# Autodesk Inventor assembly: foot
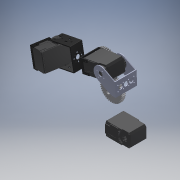
[picture p0: Inventor's stored thumbnail of the model, 180x180]
Saved by Autodesk Inventor 2019 (Build 230136000, 136)
## iProperties
Created: 2019-02-08
Part Number: foot
Document SubType Name: Assembly
Designer: mashi
Author: mashi
## iProperties of the stored document 2662N420_PLASTIC GEAR - 20 DEGREE PRESSURE ANGLE.ipt
Created: 2018-08-15
Part Number: 2662N420_PLASTIC GEAR - 20 DEGREE PRESSURE ANGLE
Material: Generic
Document SubType Name: Modeling
Designer: mashi
Density: 1 g/cm^3
Appearance: Default
Sending System: SolidWorks 2014
Last Author: T7SXC
Last Saved: 2018-08-20
Desc1: Plastic Gear—20°
Desc2: Pressure Angle
Desc3: © 2018 McMaster-Carr Supply Company
CAD Model Disclaimer and Use Terms: CAD Model Disclaimer and Use Terms.  The 3-D CAD models and related information are provided for reference only.  Your use of the CAD models is at your own risk and McMaster-Carr shall have no liability for such use.  McMaster-Carr makes no representation or warranty (express or implied) with respect to the CAD Models.  In addition, by downloading and/or using the CAD models, you agree to McMaster-Carr’s Terms and Conditions of Use and Sale, available at our website as follows: https://www.mcmaster.com/#termsandconditions
Author: mashi
## iProperties of the stored document bracketadapter2.ipt
Created: 2018-10-09
Part Number: bracketadapter2
Material: Generic
Document SubType Name: Modeling
Designer: mashi
Density: 1 g/cm^3
Appearance: Default
Sending System: SolidWorks 2018
Last Author: chang
Last Saved: 2018-10-09
Author: mashi
## iProperties of the stored document 90 Degree Servo Bracket.ipt
Created: 2018-10-07
Part Number: 90 Degree Servo Bracket
Material: Generic
Document SubType Name: Modeling
Designer: mashi
Density: 1 g/cm^3
Appearance: Default
Sending System: SolidWorks 2016
Last Author: henri
Last Saved: 2018-10-07
Author: mashi
## iProperties of the stored document Servo Motor Front Bracket.ipt
Created: 2018-10-07
Part Number: Servo Motor Front Bracket
Material: Generic
Document SubType Name: Modeling
Designer: mashi
Density: 1 g/cm^3
Appearance: Default
Sending System: SolidWorks 2018
Last Author: HP
Last Saved: 2018-10-09
Author: mashi
## iProperties of the stored document 45 Degree Servo Bracket.ipt
Created: 2018-09-28
Part Number: 45 Degree Servo Bracket
Material: Generic
Document SubType Name: Modeling
Designer: mashi
Density: 1 g/cm^3
Appearance: Default
Sending System: SolidWorks 2018
Last Author: yz3400
Last Saved: 2018-10-12
Author: mashi
## iProperties of the stored document Lewansoul LX-16A Servo.ipt
Created: 2018-10-09
Part Number: Lewansoul LX-16A Servo
Material: Generic
Description: Rhino converted to STEP
Document SubType Name: Modeling
Designer: mashi
Density: 1 g/cm^3
Appearance: Default
Sending System: SolidWorks 2018
Last Author: chang
Last Saved: 2018-10-09
Nomenclature: Document
Part Number: Document
Source: MADE
Definition: A
Author: mashi
Revision Number: A
## iProperties of the stored document Servo Motor Side Bracket.ipt
Created: 2018-10-08
Part Number: Servo Motor Side Bracket
Material: Generic
Document SubType Name: Modeling
Designer: mashi
Density: 1 g/cm^3
Appearance: Default
Sending System: SolidWorks 2018
Last Author: admin
Last Saved: 2018-10-08
Author: mashi
## iProperties of the stored document bracketadapter1.ipt
Created: 2018-10-09
Part Number: bracketadapter1
Material: Generic
Document SubType Name: Modeling
Designer: mashi
Density: 1 g/cm^3
Appearance: Default
Sending System: SolidWorks 2018
Last Author: chang
Last Saved: 2018-10-26
Author: mashi
## Documents named in this file (17)
- **C:\Users\mashi\Desktop\Robotics Studio\Rollbot\foot.iam*LocalDocs*xMgcmj2lsNkefe0wdXyyahf42Mc*2662N420_PLASTIC GEAR - 20 DEGREE PRESSURE ANGLE.ipt
- **C:\Users\mashi\Desktop\Robotics Studio\Rollbot\foot.iam*LocalDocs*x5lasmzqhNc3iev4mMcwajm4oAd*bracketadapter2.ipt
- **C:\Users\mashi\Desktop\Robotics Studio\Rollbot\foot.iam*LocalDocs*x1hcrqoyvZnlvu3kpF2lxyrgt4f*90 Degree Servo Bracket.ipt
- **C:\Users\mashi\Desktop\Robotics Studio\Rollbot\foot.iam*LocalDocs*xLrj4xvnuB5roujkdXhhuxaueNh*Servo Motor Front Bracket.ipt
- **C:\Users\mashi\Desktop\Robotics Studio\Rollbot\foot.iam*LocalDocs*xTrqjmq2aYiq3umchNmrlfejoAg*45 Degree Servo Bracket.ipt
- **C:\Users\mashi\Desktop\Robotics Studio\Rollbot\foot.iam*LocalDocs*xRjd4zsbt1wuze3ohJqu54l3rWh*Lewansoul LX-16A Servo.ipt
- **C:\Users\mashi\Desktop\Robotics Studio\Rollbot\foot.iam*LocalDocs*xVpqaq2tw5ebsussnJvcm3i000d*Servo Motor Side Bracket.ipt
- **C:\Users\mashi\Desktop\Robotics Studio\Rollbot\foot.iam*LocalDocs*xWucropqwTi4ve1g5An43dijzIb*bracketadapter1.ipt
- C:\Users\mashi\Desktop\Robotics Studio\Rollbot\foot.iam
- C:\Users\mashi\Desktop\Robotics Studio\Robotics Studio___CAD Models of Electronic Components\Lewansoul LX-16A Servo.SLDPRT
- C:\Users\mashi\Desktop\Robotics Studio\Robotics Studio___CAD Models of Electronic Components\bracketadapter1.SLDPRT
- C:\Users\mashi\Desktop\Robotics Studio\Robotics Studio___CAD Models of Electronic Components\bracketadapter2.SLDPRT
- C:\Users\mashi\Desktop\Robotics Studio\Robotics Studio___CAD Models of Electronic Components\Servo Motor Front Bracket.SLDPRT
- C:\Users\mashi\Desktop\Robotics Studio\Robotics Studio___CAD Models of Electronic Components\45 Degree Servo Bracket.SLDPRT
- C:\Users\mashi\Desktop\Robotics Studio\Robotics Studio___CAD Models of Electronic Components\90 Degree Servo Bracket.SLDPRT
- C:\Users\mashi\Desktop\Robotics Studio\Robotics Studio___CAD Models of Electronic Components\Servo Motor Side Bracket.SLDPRT
- C:\Users\mashi\Desktop\Robotics Studio\Robotics Studio___CAD Models of Electronic Components\2662N420_PLASTIC GEAR - 20 DEGREE PRESSURE ANGLE.SLDPRT
## Components (14 placed, 8 different names)
1. Lewansoul LX-16A Servo:1 — Mate:1, Mate:2, Mate:3, Mate:4, Insert:1, Insert:2
2. bracketadapter1:1 — Mate:3, Mate:4
3. bracketadapter2:1 — Mate:1, Mate:2, Insert:3, Insert:4
4. Servo Motor Front Bracket:1 — Insert:1, Insert:2
5. 45 Degree Servo Bracket:1 — Insert:3, Insert:4
6. Lewansoul LX-16A Servo:2 — Mate:5, Mate:6, Insert:5, Insert:8, Insert:9
7. bracketadapter1:2 — Mate:5, Mate:6
8. bracketadapter2:2 — Insert:5, Insert:6, Insert:7
9. 90 Degree Servo Bracket:1 — Insert:6, Insert:7
10. Servo Motor Side Bracket:1 — Insert:8, Insert:9
11. 2662N420_PLASTIC GEAR - 20 DEGREE PRESSURE ANGLE:1 — Insert:10
12. 2662N420_PLASTIC GEAR - 20 DEGREE PRESSURE ANGLE:2
13. bracketadapter1:3 — Insert:10
14. Lewansoul LX-16A Servo:3
## Relationships (16: Insert 10, Mate 6)
- Mate:1: Lewansoul LX-16A Servo:1 ↔ bracketadapter2:1
- Mate:2: Lewansoul LX-16A Servo:1 ↔ bracketadapter2:1
- Mate:3: Lewansoul LX-16A Servo:1 ↔ bracketadapter1:1
- Mate:4: Lewansoul LX-16A Servo:1 ↔ bracketadapter1:1
- Insert:1: Lewansoul LX-16A Servo:1 ↔ Servo Motor Front Bracket:1
- Insert:2: Lewansoul LX-16A Servo:1 ↔ Servo Motor Front Bracket:1
- Insert:3: bracketadapter2:1 ↔ 45 Degree Servo Bracket:1
- Insert:4: bracketadapter2:1 ↔ 45 Degree Servo Bracket:1
- Mate:5: Lewansoul LX-16A Servo:2 ↔ bracketadapter1:2
- Mate:6: Lewansoul LX-16A Servo:2 ↔ bracketadapter1:2
- Insert:5: Lewansoul LX-16A Servo:2 ↔ bracketadapter2:2
- Insert:6: bracketadapter2:2 ↔ 90 Degree Servo Bracket:1
- Insert:7: bracketadapter2:2 ↔ 90 Degree Servo Bracket:1
- Insert:8: Lewansoul LX-16A Servo:2 ↔ Servo Motor Side Bracket:1
- Insert:9: Lewansoul LX-16A Servo:2 ↔ Servo Motor Side Bracket:1
- Insert:10: 2662N420_PLASTIC GEAR - 20 DEGREE PRESSURE ANGLE:1 ↔ bracketadapter1:3
